# Autodesk Inventor assembly: Backplate
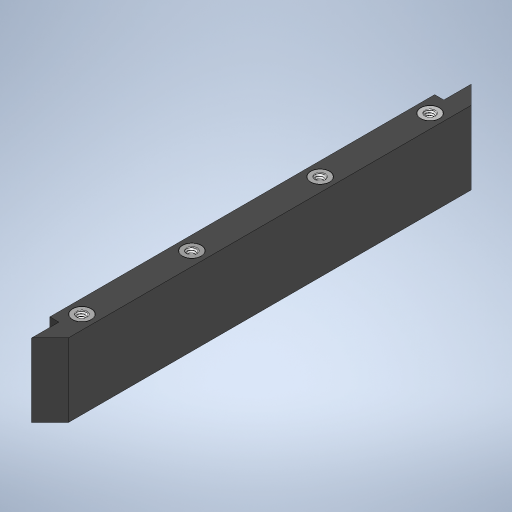
[picture p0: Inventor's stored thumbnail of the model, 512x512]
Saved by Autodesk Inventor 2023.2 (Build 272271000, 271)
## iProperties
Created: 2023-06-29
Part Number: Backplate
Document SubType Name: Assembly
Designer: Nathan Cai
Author: Nathan Cai
## Documents named in this file (3)
- E:\Documents\Inventor\Law - V1.0\Backplate.iam
- E:\Documents\Inventor\Law - V1.0\Backplate.ipt
- E:\Documents\Inventor\Law - V1.0\Standoff 1in.ipt
## Components (5 placed, 2 different names)
1. Backplate:1 — Mate:1, Mate:2, Mate:3, Mate:4, Flush:1, Flush:2, Flush:3, Flush:4
2. Standoff 1in:1 — Mate:1, Flush:1
3. Standoff 1in:2 — Mate:2, Flush:2
4. Standoff 1in:3 — Mate:3, Flush:3
5. Standoff 1in:4 — Mate:4, Flush:4
## Relationships (8: Mate 4, Flush 4)
- Mate:1: Backplate:1 ↔ Standoff 1in:1
- Mate:2: Backplate:1 ↔ Standoff 1in:2
- Mate:3: Backplate:1 ↔ Standoff 1in:3
- Mate:4: Backplate:1 ↔ Standoff 1in:4
- Flush:1: Backplate:1 ↔ Standoff 1in:1
- Flush:2: Backplate:1 ↔ Standoff 1in:2
- Flush:3: Backplate:1 ↔ Standoff 1in:3
- Flush:4: Backplate:1 ↔ Standoff 1in:4
